# Autodesk Inventor assembly: Trebuchet V1 - Assembly
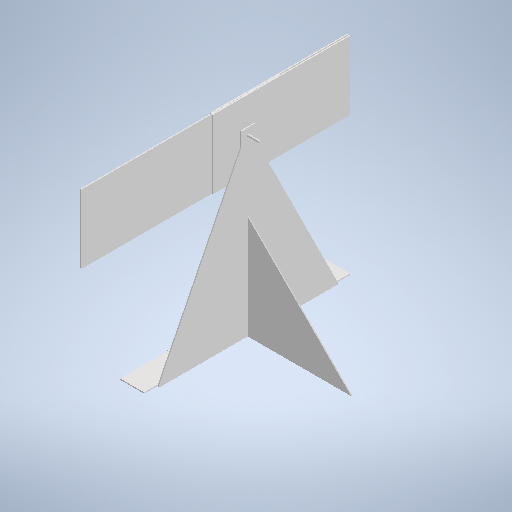
[picture p0: Inventor's stored thumbnail of the model, 512x512]
Saved by Autodesk Inventor 2025.2 (Build 292293000, 293)
## iProperties
Created: 2025-04-07
Part Number: Trebuchet V1 - Assembly
Document SubType Name: Assembly
Designer: Dylan
Author: VRK99-0110
Title: Trebuchet - Assembly
Subject: Trebuchet Project
Comments: Only half of the trebuchet was assembled so as to leave it open and viewable from all angles, making it easier to analyze and construct.
## Documents named in this file (7)
- D:\GitHub\MMAE 232\Trebuchet\V1\Trebuchet V1 - Assembly.iam
- D:\GitHub\MMAE 232\Trebuchet\V1\Trebuchet V1 - Runway.ipt
- D:\GitHub\MMAE 232\Trebuchet\V1\Trebuchet V1 - Truss.ipt
- D:\GitHub\MMAE 232\Trebuchet\V1\Trebuchet V1 - Truss Support.ipt
- D:\GitHub\MMAE 232\Trebuchet\V1\Trebuchet V1 - Long Arm (Sling).ipt
- D:\GitHub\MMAE 232\Trebuchet\V1\Trebuchet V1 - Short Arm (Weight).ipt
- D:\GitHub\MMAE 232\Trebuchet\V1\Trebuchet V1 - Acrylic Rod (78mm).ipt
## Components (7 placed, 6 different names)
1. Trebuchet V1 - Runway:1 — Mate:1, Mate:2, Flush:1
2. Trebuchet V1 - Truss:1 — Mate:1, Mate:2, Flush:1, Mate:3, Mate:4, Flush:2, Insert:4
3. Trebuchet V1 - Truss Support:1 — Mate:3, Mate:4, Flush:2
4. Trebuchet V1 - Long Arm (Sling):1 — Insert:1
5. Trebuchet V1 - Short Arm (Weight):1 — Insert:2
6. Trebuchet V1 - Acrylic Rod (78mm):1 — Insert:1, Insert:2, Insert:3, Insert:4
7. Trebuchet V1 - Short Arm (Weight):2 — Insert:3
## Relationships (10: Mate 4, Insert 4, Flush 2)
- Mate:1: Trebuchet V1 - Runway:1 ↔ Trebuchet V1 - Truss:1
- Mate:2: Trebuchet V1 - Runway:1 ↔ Trebuchet V1 - Truss:1
- Flush:1: Trebuchet V1 - Runway:1 ↔ Trebuchet V1 - Truss:1
- Mate:3: Trebuchet V1 - Truss:1 ↔ Trebuchet V1 - Truss Support:1
- Mate:4: Trebuchet V1 - Truss:1 ↔ Trebuchet V1 - Truss Support:1
- Flush:2: Trebuchet V1 - Truss:1 ↔ Trebuchet V1 - Truss Support:1
- Insert:1 (-39 mm): Trebuchet V1 - Long Arm (Sling):1 ↔ Trebuchet V1 - Acrylic Rod (78mm):1
- Insert:2 (-39 mm): Trebuchet V1 - Short Arm (Weight):1 ↔ Trebuchet V1 - Acrylic Rod (78mm):1
- Insert:3 (-35.825 mm): Trebuchet V1 - Acrylic Rod (78mm):1 ↔ Trebuchet V1 - Short Arm (Weight):2
- Insert:4 (33 mm): Trebuchet V1 - Truss:1 ↔ Trebuchet V1 - Acrylic Rod (78mm):1
